# Autodesk Inventor assembly: Level 3
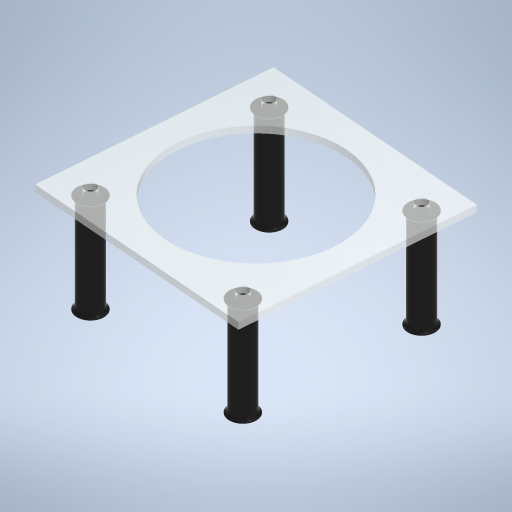
[picture p0: Inventor's stored thumbnail of the model, 512x512]
Saved by Autodesk Inventor 2024 (Build 280153000, 153)
## iProperties
Created: 2023-07-19
Part Number: Level 3
Document SubType Name: Assembly
Designer: javie
Author: javie
## Documents named in this file (3)
- C:\Users\javie\OneDrive\Documents\Inventor\L3+L4\Level 3.iam
- C:\Users\javie\OneDrive\Documents\Inventor\L3+L4\Plant Panel.ipt
- C:\Users\javie\OneDrive\Documents\Inventor\L3+L4\Top Level Pegs.ipt
## Components (5 placed, 2 different names)
1. Plant Panel:1 — Insert:1, Insert:2, Insert:3, Insert:4
2. Top Level Pegs:1 — Insert:1
3. Top Level Pegs:2 — Insert:2
4. Top Level Pegs:3 — Insert:3
5. Top Level Pegs:4 — Insert:4
## Relationships (4: Insert 4)
- Insert:1: Plant Panel:1 ↔ Top Level Pegs:1
- Insert:2: Plant Panel:1 ↔ Top Level Pegs:2
- Insert:3: Plant Panel:1 ↔ Top Level Pegs:3
- Insert:4: Plant Panel:1 ↔ Top Level Pegs:4
